# Autodesk Inventor assembly: Wind Tunnel Exhaust Frame As-built
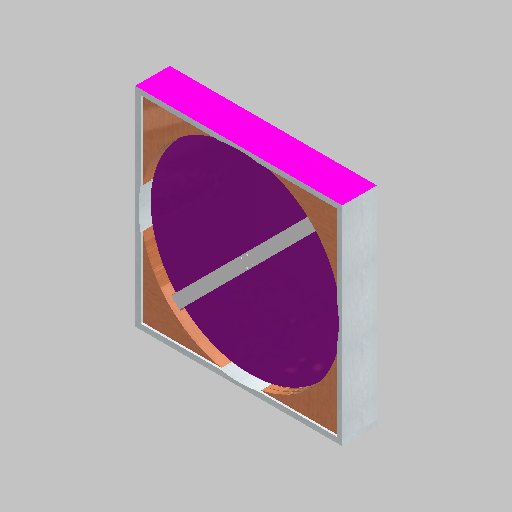
[picture p0: Inventor's stored thumbnail of the model, 512x512]
Saved by Autodesk Inventor 2023 (Build 270158000, 158)
## iProperties
Created: 2022-03-08
Part Number: Wind Tunnel Exhaust Frame As-built
Document SubType Name: Assembly
Designer: kamer
Author: kamer
## Documents named in this file (7)
- X:\Storage\Documents\ME 306 Heat Transfer Project Files\CAD\Wind Tunnel Exhaust Frame As-built.iam
- X:\Storage\Documents\ME 306 Heat Transfer Project Files\CAD\Exhaust Frame Upper+Lower as-built.ipt
- X:\Storage\Documents\ME 306 Heat Transfer Project Files\CAD\Exhaust Frame Side as built.ipt
- X:\Storage\Documents\ME 306 Heat Transfer Project Files\CAD\Wind Tunnel Fan Shroud Corner.ipt
- X:\Storage\Documents\ME 306 Heat Transfer Project Files\CAD\Propellor Close Clearance.ipt
- X:\Storage\Documents\ME 306 Heat Transfer Project Files\CAD\Wind Tunnel Fan Shroud Corner Mod Strap.ipt
- X:\Storage\Documents\ME 306 Heat Transfer Project Files\CAD\Motor Strap 5-16.ipt
## Components (30 placed, 6 different names)
1. Exhaust Frame Upper+Lower as-built:1 — Mate:2, Flush:3, Flush:4, Mate:8, Mate:11, Mate:20, Mate:23, Mate:33, Mate:34, Mate:46, Mate:47, Mate:59, Mate:62, Mate:78, Mate:81, Mate:82, Flush:13, Flush:16, Flush:17
2. Exhaust Frame Side as built:1 — Mate:2, Flush:3, Flush:4, Mate:6, Mate:10, Mate:16, Mate:21, Mate:28, Mate:35, Mate:36, Mate:42, Mate:49, Mate:54, Mate:63, Mate:68, Mate:74, Mate:79, Mate:95, Flush:14, Flush:15
3. Wind Tunnel Fan Shroud Corner:1 — Flush:8, Flush:10, Mate:13, Flush:11, Mate:94, Mate:98
4. Wind Tunnel Fan Shroud Corner:2 — Mate:8, Flush:9, Flush:10, Mate:15, Mate:83
5. Wind Tunnel Fan Shroud Corner:3 — Mate:15, Mate:23, Mate:27, Mate:84
6. Wind Tunnel Fan Shroud Corner:4 — Mate:27, Mate:33, Mate:40, Mate:85
7. Wind Tunnel Fan Shroud Corner:6 — Mate:70, Mate:89, Mate:97
8. Wind Tunnel Fan Shroud Corner:7 — Mate:40, Mate:46, Mate:53, Mate:86
9. Wind Tunnel Fan Shroud Corner:8 — Mate:53, Mate:59, Mate:72, Mate:87
10. Wind Tunnel Fan Shroud Corner:10 — Mate:51, Mate:54, Mate:71, Mate:107
11. Wind Tunnel Fan Shroud Corner:11 — Mate:41, Mate:47, Mate:49, Mate:61
12. Wind Tunnel Fan Shroud Corner:12 — Mate:39, Mate:42, Mate:51, Mate:106
13. Wind Tunnel Fan Shroud Corner:13 — Mate:38, Mate:60, Mate:91, Mate:101
14. Wind Tunnel Fan Shroud Corner:14 — Mate:26, Mate:34, Mate:35, Mate:41
15. Wind Tunnel Fan Shroud Corner:15 — Mate:25, Mate:38, Mate:92, Mate:100
16. Wind Tunnel Fan Shroud Corner:16 — Mate:24, Mate:28, Mate:39, Mate:105
17. Wind Tunnel Fan Shroud Corner:17 — Mate:14, Mate:20, Mate:21, Mate:26
18. Wind Tunnel Fan Shroud Corner:18 — Mate:13, Mate:25, Mate:93, Mate:99
19. Wind Tunnel Fan Shroud Corner:19 — Mate:12, Mate:16, Mate:24, Mate:104
20. Wind Tunnel Fan Shroud Corner:20 — Mate:10, Mate:11, Flush:9, Mate:14, Flush:17
21. Wind Tunnel Fan Shroud Corner:21 — Mate:6, Flush:8, Mate:12, Mate:103
22. Propellor Close Clearance:1 — Flush:11, Mate:36
23. Wind Tunnel Fan Shroud Corner Mod Strap:1 — Mate:60, Mate:66, Mate:70, Mate:90, Mate:91, Mate:102
24. Wind Tunnel Fan Shroud Corner Mod Strap:2 — Mate:61, Mate:62, Mate:63, Mate:73
25. Motor Strap 5-16:1 — Mate:66, Mate:68, Mate:96
26. Wind Tunnel Fan Shroud Corner:22 — Mate:73, Mate:78, Mate:79
27. Wind Tunnel Fan Shroud Corner:23 — Mate:72, Mate:81, Mate:88
28. Wind Tunnel Fan Shroud Corner:24 — Mate:71, Mate:74, Mate:108
29. Exhaust Frame Side as built:2 — Mate:82, Flush:13, Mate:83, Mate:84, Mate:85, Mate:86, Mate:87, Mate:88, Mate:89, Mate:90, Mate:92, Mate:93, Mate:94, Flush:16
30. Exhaust Frame Upper+Lower as-built:2 — Mate:95, Flush:14, Flush:15, Mate:96, Mate:97, Mate:98, Mate:99, Mate:100, Mate:101, Mate:102, Mate:103, Mate:104, Mate:105, Mate:106, Mate:107, Mate:108
## Relationships (86: Mate 75, Flush 11)
- Mate:2: Exhaust Frame Upper+Lower as-built:1 ↔ Exhaust Frame Side as built:1
- Flush:3: Exhaust Frame Upper+Lower as-built:1 ↔ Exhaust Frame Side as built:1
- Flush:4: Exhaust Frame Upper+Lower as-built:1 ↔ Exhaust Frame Side as built:1
- Mate:6: Exhaust Frame Side as built:1 ↔ Wind Tunnel Fan Shroud Corner:21
- Flush:8: Wind Tunnel Fan Shroud Corner:1 ↔ Wind Tunnel Fan Shroud Corner:21
- Mate:8: Exhaust Frame Upper+Lower as-built:1 ↔ Wind Tunnel Fan Shroud Corner:2
- Mate:10: Exhaust Frame Side as built:1 ↔ Wind Tunnel Fan Shroud Corner:20
- Mate:11: Exhaust Frame Upper+Lower as-built:1 ↔ Wind Tunnel Fan Shroud Corner:20
- Flush:9: Wind Tunnel Fan Shroud Corner:2 ↔ Wind Tunnel Fan Shroud Corner:20
- Flush:10: Wind Tunnel Fan Shroud Corner:1 ↔ Wind Tunnel Fan Shroud Corner:2
- Mate:12: Wind Tunnel Fan Shroud Corner:19 ↔ Wind Tunnel Fan Shroud Corner:21
- Mate:13: Wind Tunnel Fan Shroud Corner:1 ↔ Wind Tunnel Fan Shroud Corner:18
- Mate:14: Wind Tunnel Fan Shroud Corner:17 ↔ Wind Tunnel Fan Shroud Corner:20
- Mate:15: Wind Tunnel Fan Shroud Corner:2 ↔ Wind Tunnel Fan Shroud Corner:3
- Mate:16: Exhaust Frame Side as built:1 ↔ Wind Tunnel Fan Shroud Corner:19
- Mate:20: Exhaust Frame Upper+Lower as-built:1 ↔ Wind Tunnel Fan Shroud Corner:17
- Mate:21: Exhaust Frame Side as built:1 ↔ Wind Tunnel Fan Shroud Corner:17
- Mate:23: Exhaust Frame Upper+Lower as-built:1 ↔ Wind Tunnel Fan Shroud Corner:3
- Mate:24: Wind Tunnel Fan Shroud Corner:16 ↔ Wind Tunnel Fan Shroud Corner:19
- Mate:25: Wind Tunnel Fan Shroud Corner:15 ↔ Wind Tunnel Fan Shroud Corner:18
- Mate:26: Wind Tunnel Fan Shroud Corner:14 ↔ Wind Tunnel Fan Shroud Corner:17
- Mate:27: Wind Tunnel Fan Shroud Corner:3 ↔ Wind Tunnel Fan Shroud Corner:4
- Mate:28: Exhaust Frame Side as built:1 ↔ Wind Tunnel Fan Shroud Corner:16
- Mate:33: Exhaust Frame Upper+Lower as-built:1 ↔ Wind Tunnel Fan Shroud Corner:4
- Mate:34: Exhaust Frame Upper+Lower as-built:1 ↔ Wind Tunnel Fan Shroud Corner:14
- Mate:35: Exhaust Frame Side as built:1 ↔ Wind Tunnel Fan Shroud Corner:14
- Flush:11: Wind Tunnel Fan Shroud Corner:1 ↔ Propellor Close Clearance:1
- Mate:36 (215.8683 mm): Exhaust Frame Side as built:1 ↔ Propellor Close Clearance:1
- Mate:38: Wind Tunnel Fan Shroud Corner:13 ↔ Wind Tunnel Fan Shroud Corner:15
- Mate:39: Wind Tunnel Fan Shroud Corner:12 ↔ Wind Tunnel Fan Shroud Corner:16
- Mate:40: Wind Tunnel Fan Shroud Corner:4 ↔ Wind Tunnel Fan Shroud Corner:7
- Mate:41: Wind Tunnel Fan Shroud Corner:11 ↔ Wind Tunnel Fan Shroud Corner:14
- Mate:42: Exhaust Frame Side as built:1 ↔ Wind Tunnel Fan Shroud Corner:12
- Mate:46: Exhaust Frame Upper+Lower as-built:1 ↔ Wind Tunnel Fan Shroud Corner:7
- Mate:47: Exhaust Frame Upper+Lower as-built:1 ↔ Wind Tunnel Fan Shroud Corner:11
- Mate:49: Exhaust Frame Side as built:1 ↔ Wind Tunnel Fan Shroud Corner:11
- Mate:51: Wind Tunnel Fan Shroud Corner:10 ↔ Wind Tunnel Fan Shroud Corner:12
- Mate:53: Wind Tunnel Fan Shroud Corner:7 ↔ Wind Tunnel Fan Shroud Corner:8
- Mate:54: Exhaust Frame Side as built:1 ↔ Wind Tunnel Fan Shroud Corner:10
- Mate:59: Exhaust Frame Upper+Lower as-built:1 ↔ Wind Tunnel Fan Shroud Corner:8
- Mate:60: Wind Tunnel Fan Shroud Corner:13 ↔ Wind Tunnel Fan Shroud Corner Mod Strap:1
- Mate:61: Wind Tunnel Fan Shroud Corner:11 ↔ Wind Tunnel Fan Shroud Corner Mod Strap:2
- Mate:62: Exhaust Frame Upper+Lower as-built:1 ↔ Wind Tunnel Fan Shroud Corner Mod Strap:2
- Mate:63: Exhaust Frame Side as built:1 ↔ Wind Tunnel Fan Shroud Corner Mod Strap:2
- Mate:66: Wind Tunnel Fan Shroud Corner Mod Strap:1 ↔ Motor Strap 5-16:1
- Mate:68: Exhaust Frame Side as built:1 ↔ Motor Strap 5-16:1
- Mate:70: Wind Tunnel Fan Shroud Corner:6 ↔ Wind Tunnel Fan Shroud Corner Mod Strap:1
- Mate:71: Wind Tunnel Fan Shroud Corner:10 ↔ Wind Tunnel Fan Shroud Corner:24
- Mate:72: Wind Tunnel Fan Shroud Corner:8 ↔ Wind Tunnel Fan Shroud Corner:23
- Mate:73: Wind Tunnel Fan Shroud Corner Mod Strap:2 ↔ Wind Tunnel Fan Shroud Corner:22
- Mate:74: Exhaust Frame Side as built:1 ↔ Wind Tunnel Fan Shroud Corner:24
- Mate:78: Exhaust Frame Upper+Lower as-built:1 ↔ Wind Tunnel Fan Shroud Corner:22
- Mate:79: Exhaust Frame Side as built:1 ↔ Wind Tunnel Fan Shroud Corner:22
- Mate:81: Exhaust Frame Upper+Lower as-built:1 ↔ Wind Tunnel Fan Shroud Corner:23
- Mate:82: Exhaust Frame Upper+Lower as-built:1 ↔ Exhaust Frame Side as built:2
- Flush:13: Exhaust Frame Upper+Lower as-built:1 ↔ Exhaust Frame Side as built:2
- Mate:83: Wind Tunnel Fan Shroud Corner:2 ↔ Exhaust Frame Side as built:2
- Mate:84: Wind Tunnel Fan Shroud Corner:3 ↔ Exhaust Frame Side as built:2
- Mate:85: Wind Tunnel Fan Shroud Corner:4 ↔ Exhaust Frame Side as built:2
- Mate:86: Wind Tunnel Fan Shroud Corner:7 ↔ Exhaust Frame Side as built:2
- Mate:87: Wind Tunnel Fan Shroud Corner:8 ↔ Exhaust Frame Side as built:2
- Mate:88: Wind Tunnel Fan Shroud Corner:23 ↔ Exhaust Frame Side as built:2
- Mate:89: Wind Tunnel Fan Shroud Corner:6 ↔ Exhaust Frame Side as built:2
- Mate:90: Wind Tunnel Fan Shroud Corner Mod Strap:1 ↔ Exhaust Frame Side as built:2
- Mate:91: Wind Tunnel Fan Shroud Corner:13 ↔ Wind Tunnel Fan Shroud Corner Mod Strap:1
- Mate:92: Wind Tunnel Fan Shroud Corner:15 ↔ Exhaust Frame Side as built:2
- Mate:93: Wind Tunnel Fan Shroud Corner:18 ↔ Exhaust Frame Side as built:2
- Mate:94: Wind Tunnel Fan Shroud Corner:1 ↔ Exhaust Frame Side as built:2
- Mate:95: Exhaust Frame Side as built:1 ↔ Exhaust Frame Upper+Lower as-built:2
- Flush:14: Exhaust Frame Side as built:1 ↔ Exhaust Frame Upper+Lower as-built:2
- Flush:15: Exhaust Frame Side as built:1 ↔ Exhaust Frame Upper+Lower as-built:2
- Flush:16: Exhaust Frame Upper+Lower as-built:1 ↔ Exhaust Frame Side as built:2
- Flush:17: Exhaust Frame Upper+Lower as-built:1 ↔ Wind Tunnel Fan Shroud Corner:20
- Mate:96: Motor Strap 5-16:1 ↔ Exhaust Frame Upper+Lower as-built:2
- Mate:97: Wind Tunnel Fan Shroud Corner:6 ↔ Exhaust Frame Upper+Lower as-built:2
- Mate:98: Wind Tunnel Fan Shroud Corner:1 ↔ Exhaust Frame Upper+Lower as-built:2
- Mate:99: Wind Tunnel Fan Shroud Corner:18 ↔ Exhaust Frame Upper+Lower as-built:2
- Mate:100: Wind Tunnel Fan Shroud Corner:15 ↔ Exhaust Frame Upper+Lower as-built:2
- Mate:101: Wind Tunnel Fan Shroud Corner:13 ↔ Exhaust Frame Upper+Lower as-built:2
- Mate:102: Wind Tunnel Fan Shroud Corner Mod Strap:1 ↔ Exhaust Frame Upper+Lower as-built:2
- Mate:103: Wind Tunnel Fan Shroud Corner:21 ↔ Exhaust Frame Upper+Lower as-built:2
- Mate:104: Wind Tunnel Fan Shroud Corner:19 ↔ Exhaust Frame Upper+Lower as-built:2
- Mate:105: Wind Tunnel Fan Shroud Corner:16 ↔ Exhaust Frame Upper+Lower as-built:2
- Mate:106: Wind Tunnel Fan Shroud Corner:12 ↔ Exhaust Frame Upper+Lower as-built:2
- Mate:107: Wind Tunnel Fan Shroud Corner:10 ↔ Exhaust Frame Upper+Lower as-built:2
- Mate:108: Wind Tunnel Fan Shroud Corner:24 ↔ Exhaust Frame Upper+Lower as-built:2
